# Autodesk Inventor assembly: POM_T5_13
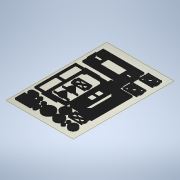
[picture p0: Inventor's stored thumbnail of the model, 180x180]
Saved by Autodesk Inventor 2020 (Build 240168000, 168)
## iProperties
Created: 2021-08-27
Part Number: POM_T5_13
Document SubType Name: Assembly
Designer: Masato
Author: Masato
## Documents named in this file (20)
- C:\Inventor\SUSTAINA-OP\Cam\POM_T5_13.iam
- C:\Inventor\SUSTAINA-OP\Cam\DisposableBoard.ipt
- C:\Inventor\SUSTAINA-OP\SandBlastingJig\Foot_front_frame_SandBlastingJig_back.ipt
- C:\Inventor\SUSTAINA-OP\SandBlastingJig\Foot_front_frame_SandBlastingJig_front.ipt
- C:\Inventor\SUSTAINA-OP\SandBlastingJig\Leg_joint_slider_frame_SandBlastingJig_axis_back.ipt
- C:\Inventor\SUSTAINA-OP\SandBlastingJig\Leg_joint_slider_frame_SandBlastingJig_axis_front.ipt
- C:\Inventor\SUSTAINA-OP\SandBlastingJig\Leg_joint_slider_frame_SandBlastingJig_slider_back.ipt
- C:\Inventor\SUSTAINA-OP\SandBlastingJig\Leg_joint_slider_frame_SandBlastingJig_slider_front.ipt
- C:\Inventor\SUSTAINA-OP\SandBlastingJig\Leg_joint_yaw_frame_SandBlastingJig.ipt
- C:\Inventor\SUSTAINA-OP\SandBlastingJig\Outer_support_stand_SandBlastingJig.ipt
- C:\Inventor\SUSTAINA-OP\SandBlastingJig\Shoulder_horn_frame_SandBlastingJig.ipt
- C:\Inventor\SUSTAINA-OP\SandBlastingJig\Trunk_neck_frame_AND_Trunk_shoulder_frame_SandBlastingJig.ipt
- C:\Inventor\SUSTAINA-OP\SandBlastingJig\Trunk_servo_bottom_frame_SandBlastingJig.ipt
- C:\Inventor\SUSTAINA-OP\UpperBody\Cockpit\Cockpit_circuit_board_frame.ipt
- C:\Inventor\SUSTAINA-OP\UpperBody\Cockpit\Cockpit_back_frame.ipt
- C:\Inventor\SUSTAINA-OP\UpperBody\Cockpit\Cockpit_battery_back_door.ipt
- C:\Inventor\SUSTAINA-OP\UpperBody\Cockpit\Cockpit_top_frame.ipt
- C:\Inventor\SUSTAINA-OP\UpperBody\Head\Head_horn_frame.ipt
- C:\Inventor\SUSTAINA-OP\UpperBody\Head\Camera_side_frame.ipt
- C:\Inventor\SUSTAINA-OP\UpperBody\Head\Head_diagonal.ipt
## Components (22 placed, 19 different names)
1. DisposableBoard:1 — メイト:2, メイト:1, フラッシュ:1, フラッシュ:2, メイト:13, メイト:15, メイト:16, メイト:17, メイト:18, メイト:19, メイト:20, メイト:21, メイト:22, メイト:23, 角度:1, 角度:3, 角度:4, 角度:5, 角度:6, 角度:7, フラッシュ:3, フラッシュ:4, 正接:20, 正接:25, 正接:27, 正接:30, 角度:8, メイト:35, 角度:9, メイト:36, メイト:38, メイト:39, フラッシュ:5, メイト:41, メイト:45, メイト:49, メイト:52, メイト:54
2. Foot_front_frame_SandBlastingJig_back:1 — メイト:22, 角度:4, 正接:22, 正接:23
3. Foot_front_frame_SandBlastingJig_front:1 — メイト:23, 角度:5, 正接:14, 正接:15
4. Leg_joint_slider_frame_SandBlastingJig_axis_back:1 — メイト:18, 角度:7, 正接:19, 正接:26, 正接:27
5. Leg_joint_slider_frame_SandBlastingJig_axis_front:1 — メイト:15, 角度:6, 正接:19, 正接:28, 正接:29
6. Leg_joint_slider_frame_SandBlastingJig_slider_back:1 — メイト:17, メイト:34, 正接:2, 正接:4, 正接:14
7. Leg_joint_slider_frame_SandBlastingJig_slider_front:1 — メイト:19, メイト:33, 正接:20, 正接:22, メイト:40
8. Leg_joint_yaw_frame_SandBlastingJig:1 — メイト:20, 正接:29, 正接:30, 角度:8
9. Outer_support_stand_SandBlastingJig:1 — メイト:16, 角度:1, 正接:3, 正接:4, 正接:24, 正接:32
10. Shoulder_horn_frame_SandBlastingJig:1 — メイト:21, 角度:3, 正接:24, 正接:25, 正接:26, 正接:28, 正接:31
11. Trunk_servo_bottom_frame_SandBlastingJig:1 — メイト:13, メイト:33, メイト:34, 正接:2, 正接:3, 正接:15, フラッシュ:3, フラッシュ:4, 正接:23
12. Trunk_neck_frame_AND_Trunk_shoulder_frame_SandBlastingJig:1 — メイト:35, 角度:9, 正接:31, 正接:32, 正接:33, 正接:34, 正接:36
13. Cockpit_circuit_board_frame:1 — メイト:39, フラッシュ:5, 正接:33, メイト:40, フラッシュ:6, メイト:42, フラッシュ:7, メイト:50, メイト:51, メイト:53
14. Cockpit_back_frame:1 — メイト:38, フラッシュ:7, メイト:44, メイト:47, メイト:48
15. Cockpit_battery_back_door:1 — メイト:36, フラッシュ:6, メイト:43, メイト:55
16. Cockpit_top_frame:1 — メイト:41, メイト:42, メイト:43, 正接:34, メイト:44
17. Head_diagonal:1 — メイト:52, 正接:35, メイト:53
18. Head_diagonal:2 — メイト:54, メイト:55, 正接:36
19. Head_horn_frame:1 — メイト:45, メイト:47, メイト:48
20. Head_horn_frame:2
21. Camera_side_frame:2 — メイト:49, メイト:50, メイト:51
22. Camera_side_frame:3 — 正接:35
## Component patterns: (2 elements, first: Head_horn_frame:1), (2 elements, first: Camera_side_frame:2)
## Relationships (70: Mate 33, Tangent 22, Angle 8, Flush 7)
- メイト:2 [Mate]: DisposableBoard:1
- メイト:1 [Mate]: DisposableBoard:1
- フラッシュ:1 [Flush]: DisposableBoard:1
- フラッシュ:2 [Flush]: DisposableBoard:1
- メイト:13 [Mate]: DisposableBoard:1 ↔ Trunk_servo_bottom_frame_SandBlastingJig:1
- メイト:15 [Mate]: DisposableBoard:1 ↔ Leg_joint_slider_frame_SandBlastingJig_axis_front:1
- メイト:16 [Mate]: DisposableBoard:1 ↔ Outer_support_stand_SandBlastingJig:1
- メイト:17 [Mate]: DisposableBoard:1 ↔ Leg_joint_slider_frame_SandBlastingJig_slider_back:1
- メイト:18 [Mate]: DisposableBoard:1 ↔ Leg_joint_slider_frame_SandBlastingJig_axis_back:1
- メイト:19 [Mate]: DisposableBoard:1 ↔ Leg_joint_slider_frame_SandBlastingJig_slider_front:1
- メイト:20 [Mate]: DisposableBoard:1 ↔ Leg_joint_yaw_frame_SandBlastingJig:1
- メイト:21 [Mate]: DisposableBoard:1 ↔ Shoulder_horn_frame_SandBlastingJig:1
- メイト:22 [Mate]: DisposableBoard:1 ↔ Foot_front_frame_SandBlastingJig_back:1
- メイト:23 [Mate]: DisposableBoard:1 ↔ Foot_front_frame_SandBlastingJig_front:1
- メイト:33 [Mate] (2.5 mm): Leg_joint_slider_frame_SandBlastingJig_slider_front:1 ↔ Trunk_servo_bottom_frame_SandBlastingJig:1
- メイト:34 [Mate] (2.5 mm): Leg_joint_slider_frame_SandBlastingJig_slider_back:1 ↔ Trunk_servo_bottom_frame_SandBlastingJig:1
- 正接:2 [Tangent]: Leg_joint_slider_frame_SandBlastingJig_slider_back:1 ↔ Trunk_servo_bottom_frame_SandBlastingJig:1
- 角度:1 [Angle] (0 deg): DisposableBoard:1 ↔ Outer_support_stand_SandBlastingJig:1
- 正接:3 [Tangent]: Outer_support_stand_SandBlastingJig:1 ↔ Trunk_servo_bottom_frame_SandBlastingJig:1
- 正接:4 [Tangent] (2.5 mm): Leg_joint_slider_frame_SandBlastingJig_slider_back:1 ↔ Outer_support_stand_SandBlastingJig:1
- 角度:3 [Angle] (0 deg): DisposableBoard:1 ↔ Shoulder_horn_frame_SandBlastingJig:1
- 角度:4 [Angle] (0 deg): DisposableBoard:1 ↔ Foot_front_frame_SandBlastingJig_back:1
- 角度:5 [Angle] (0 deg): DisposableBoard:1 ↔ Foot_front_frame_SandBlastingJig_front:1
- 正接:14 [Tangent] (2.5 mm): Foot_front_frame_SandBlastingJig_front:1 ↔ Leg_joint_slider_frame_SandBlastingJig_slider_back:1
- 正接:15 [Tangent] (2.5 mm): Foot_front_frame_SandBlastingJig_front:1 ↔ Trunk_servo_bottom_frame_SandBlastingJig:1
- 角度:6 [Angle] (0 deg): DisposableBoard:1 ↔ Leg_joint_slider_frame_SandBlastingJig_axis_front:1
- 角度:7 [Angle] (0 deg): DisposableBoard:1 ↔ Leg_joint_slider_frame_SandBlastingJig_axis_back:1
- 正接:19 [Tangent] (2.5 mm): Leg_joint_slider_frame_SandBlastingJig_axis_back:1 ↔ Leg_joint_slider_frame_SandBlastingJig_axis_front:1
- フラッシュ:3 [Flush] (2 mm): DisposableBoard:1 ↔ Trunk_servo_bottom_frame_SandBlastingJig:1
- フラッシュ:4 [Flush] (2 mm): DisposableBoard:1 ↔ Trunk_servo_bottom_frame_SandBlastingJig:1
- 正接:20 [Tangent] (2 mm): DisposableBoard:1 ↔ Leg_joint_slider_frame_SandBlastingJig_slider_front:1
- 正接:22 [Tangent] (2.5 mm): Foot_front_frame_SandBlastingJig_back:1 ↔ Leg_joint_slider_frame_SandBlastingJig_slider_front:1
- 正接:23 [Tangent] (2.5 mm): Foot_front_frame_SandBlastingJig_back:1 ↔ Trunk_servo_bottom_frame_SandBlastingJig:1
- 正接:24 [Tangent] (2.5 mm): Outer_support_stand_SandBlastingJig:1 ↔ Shoulder_horn_frame_SandBlastingJig:1
- 正接:25 [Tangent] (2 mm): DisposableBoard:1 ↔ Shoulder_horn_frame_SandBlastingJig:1
- 正接:26 [Tangent] (2.5 mm): Leg_joint_slider_frame_SandBlastingJig_axis_back:1 ↔ Shoulder_horn_frame_SandBlastingJig:1
- 正接:27 [Tangent] (2 mm): DisposableBoard:1 ↔ Leg_joint_slider_frame_SandBlastingJig_axis_back:1
- 正接:28 [Tangent] (2.5 mm): Leg_joint_slider_frame_SandBlastingJig_axis_front:1 ↔ Shoulder_horn_frame_SandBlastingJig:1
- 正接:29 [Tangent] (2.5 mm): Leg_joint_slider_frame_SandBlastingJig_axis_front:1 ↔ Leg_joint_yaw_frame_SandBlastingJig:1
- 正接:30 [Tangent] (2 mm): DisposableBoard:1 ↔ Leg_joint_yaw_frame_SandBlastingJig:1
- 角度:8 [Angle] (0 deg): DisposableBoard:1 ↔ Leg_joint_yaw_frame_SandBlastingJig:1
- メイト:35 [Mate]: DisposableBoard:1 ↔ Trunk_neck_frame_AND_Trunk_shoulder_frame_SandBlastingJig:1
- 角度:9 [Angle] (0 deg): DisposableBoard:1 ↔ Trunk_neck_frame_AND_Trunk_shoulder_frame_SandBlastingJig:1
- 正接:31 [Tangent] (2.5 mm): Shoulder_horn_frame_SandBlastingJig:1 ↔ Trunk_neck_frame_AND_Trunk_shoulder_frame_SandBlastingJig:1
- 正接:32 [Tangent] (2.5 mm): Outer_support_stand_SandBlastingJig:1 ↔ Trunk_neck_frame_AND_Trunk_shoulder_frame_SandBlastingJig:1
- メイト:36 [Mate]: DisposableBoard:1 ↔ Cockpit_battery_back_door:1
- メイト:38 [Mate]: DisposableBoard:1 ↔ Cockpit_back_frame:1
- メイト:39 [Mate]: DisposableBoard:1 ↔ Cockpit_circuit_board_frame:1
- フラッシュ:5 [Flush] (2 mm): DisposableBoard:1 ↔ Cockpit_circuit_board_frame:1
- 正接:33 [Tangent] (2.5 mm): Trunk_neck_frame_AND_Trunk_shoulder_frame_SandBlastingJig:1 ↔ Cockpit_circuit_board_frame:1
- メイト:40 [Mate] (4.072 mm): Leg_joint_slider_frame_SandBlastingJig_slider_front:1 ↔ Cockpit_circuit_board_frame:1
- フラッシュ:6 [Flush]: Cockpit_circuit_board_frame:1 ↔ Cockpit_battery_back_door:1
- メイト:41 [Mate]: DisposableBoard:1 ↔ Cockpit_top_frame:1
- メイト:42 [Mate] (2.5 mm): Cockpit_circuit_board_frame:1 ↔ Cockpit_top_frame:1
- メイト:43 [Mate] (2.5 mm): Cockpit_battery_back_door:1 ↔ Cockpit_top_frame:1
- 正接:34 [Tangent] (2.5 mm): Trunk_neck_frame_AND_Trunk_shoulder_frame_SandBlastingJig:1 ↔ Cockpit_top_frame:1
- フラッシュ:7 [Flush]: Cockpit_circuit_board_frame:1 ↔ Cockpit_back_frame:1
- メイト:44 [Mate] (2.5 mm): Cockpit_back_frame:1 ↔ Cockpit_top_frame:1
- メイト:45 [Mate]: DisposableBoard:1 ↔ Head_horn_frame:1
- メイト:47 [Mate] (2.5 mm): Cockpit_back_frame:1 ↔ Head_horn_frame:1
- メイト:48 [Mate] (2.5 mm): Cockpit_back_frame:1 ↔ Head_horn_frame:1
- メイト:49 [Mate]: DisposableBoard:1 ↔ Camera_side_frame:2
- メイト:50 [Mate] (7 mm): Cockpit_circuit_board_frame:1 ↔ Camera_side_frame:2
- メイト:51 [Mate] (6 mm): Cockpit_circuit_board_frame:1 ↔ Camera_side_frame:2
- メイト:52 [Mate]: DisposableBoard:1 ↔ Head_diagonal:1
- 正接:35 [Tangent] (2.5 mm): Head_diagonal:1 ↔ Camera_side_frame:3
- メイト:53 [Mate] (7 mm): Cockpit_circuit_board_frame:1 ↔ Head_diagonal:1
- メイト:54 [Mate]: DisposableBoard:1 ↔ Head_diagonal:2
- メイト:55 [Mate] (2.5 mm): Cockpit_battery_back_door:1 ↔ Head_diagonal:2
- 正接:36 [Tangent] (2.5 mm): Trunk_neck_frame_AND_Trunk_shoulder_frame_SandBlastingJig:1 ↔ Head_diagonal:2
